# Autodesk Inventor assembly: roller-limit-switch
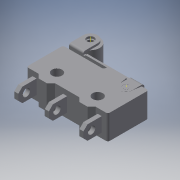
[picture p0: Inventor's stored thumbnail of the model, 180x180]
Saved by Autodesk Inventor 2018 (Build 220112000, 112)
## iProperties
Created: 2017-11-12
Part Number: roller-limit-switch
Document SubType Name: Assembly
Designer: leo2a
Author: leo2a
## Documents named in this file (5)
- C:\Users\leo2a\Documents\inventor-models\sensors\roller-limit-switch\roller-limit-switch.iam
- C:\Users\leo2a\Documents\inventor-models\sensors\roller-limit-switch\body.ipt
- C:\Users\leo2a\Documents\inventor-models\sensors\roller-limit-switch\paddle.ipt
- C:\Users\leo2a\Documents\inventor-models\sensors\roller-limit-switch\roller.ipt
- C:\Users\leo2a\Documents\inventor-models\sensors\roller-limit-switch\roller-limit-switch\Design Accelerator\Cross Pin Connection1.iam
## Components (4 placed, 4 different names)
1. body:1 — Flush:1, Mate:2
2. paddle:1 — Flush:1, Mate:1, Mate:3, Mate:4
3. roller:1 — Flush:2, Mate:5
4. Cross Pin Connection:1 [sub-assembly] — Mate:4, Mate:5
## Relationships (8: Mate 5, Flush 2, Angle 1)
- Flush:1: body:1 ↔ paddle:1
- Mate:1: paddle:1
- Mate:2: body:1
- Mate:3: paddle:1
- Angle:1 (0 deg)
- Flush:2: roller:1
- Mate:4: paddle:1 ↔ Cross Pin Connection:1
- Mate:5: roller:1 ↔ Cross Pin Connection:1
